# Autodesk Inventor assembly: FinalShooterStorage-ver2-1111-2021
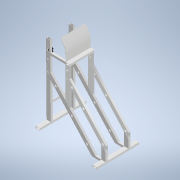
[picture p0: Inventor's stored thumbnail of the model, 180x180]
Saved by Autodesk Inventor 2021 (Build 250183000, 183)
## iProperties
Created: 2021-03-18
Part Number: FinalShooterStorage-ver2-1111-2021
Document SubType Name: Assembly
Designer: CMurray
Author: CMurray
## Documents named in this file (3)
- F:\PHRC CADD 2021\PHRC CADD\2020 Infinite Recharge\Storage\Assemblies\FinalShooterStorage-ver2-1111-2021.iam
- F:\PHRC CADD 2021\PHRC CADD\2020 Infinite Recharge\Storage\Assemblies\StorageAssembly-ver6-1111-2021.iam
- F:\PHRC CADD 2021\PHRC CADD\2020 Infinite Recharge\Shooting\Assemblies\ShooterPrototype-ver4-1111-2021.iam
## Components (2 placed, 2 different names)
1. StorageAssembly-ver6-1111-2021:1 [sub-assembly] — Mate:1, Flush:1, Mate:2
2. ShooterPrototype-ver4-1111-2021:1 [sub-assembly] — Mate:1, Flush:1, Mate:2
## Relationships (3: Mate 2, Flush 1)
- Mate:1: StorageAssembly-ver6-1111-2021:1 ↔ ShooterPrototype-ver4-1111-2021:1
- Flush:1: StorageAssembly-ver6-1111-2021:1 ↔ ShooterPrototype-ver4-1111-2021:1
- Mate:2 (459.0034 mm): StorageAssembly-ver6-1111-2021:1 ↔ ShooterPrototype-ver4-1111-2021:1
